# Autodesk Inventor assembly: YAxisMotorRight
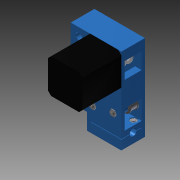
[picture p0: Inventor's stored thumbnail of the model, 180x180]
Saved by Autodesk Inventor 2015 SP1 (Build 190203100, 203)
## iProperties
Created: 2014-08-15
Part Number: YAxisMotorRight
Document SubType Name: Assembly
Designer: Jack
Mass: 240.117 g
Surface Area: 676.48 cm^2
Volume: 180.958 cm^3
Density: 1.32692 g/cm^3
Author: Jack
Title: Y Motor Right
## Documents named in this file (16)
- C:\Users\Jack\ownCloud\Projects\CrossBot\InventorModel\YAxis\YAxisMotorRight.iam
- C:\Users\Jack\ownCloud\Projects\CrossBot\InventorModel\YAxis\YAxisMotor\YMotorBlockRight.ipt
- C:\Users\Jack\ownCloud\Projects\CrossBot\InventorModel\YAxis\YAxisMotor\YMotorCapRight.ipt
- C:\Users\Jack\ownCloud\Projects\CrossBot\InventorModel\Hardware\Bolts\SHCS\SHCS4\SHCS4x30.ipt
- C:\Users\Jack\ownCloud\Projects\CrossBot\InventorModel\Hardware\Bolts\SHCS\SHCS3\SHCS3x8.ipt
- C:\Users\Jack\ownCloud\Projects\CrossBot\InventorModel\Hardware\Bearing\BearingRadialBall\BearingRadialBallF624zz.ipt
- C:\Users\Jack\ownCloud\Projects\CrossBot\InventorModel\Hardware\Wahsers\M4Washer.ipt
- C:\Users\Jack\ownCloud\Projects\CrossBot\InventorModel\Hardware\Nuts\Nut4.ipt
- C:\Users\Jack\ownCloud\Projects\CrossBot\InventorModel\Hardware\Bolts\SHCS\SHCS4\SHCS4x15.ipt
- C:\Users\Jack\ownCloud\Projects\CrossBot\InventorModel\YAxis\YAxisBearingSpacer.ipt
- C:\Users\Jack\ownCloud\Projects\CrossBot\InventorModel\Electronics\Motors\StepperMotorNema17x48mm.ipt
- C:\Users\Jack\ownCloud\Projects\CrossBot\InventorModel\Hardware\Belt\PulleyGT2x36x5Bore.ipt
- C:\Users\Jack\ownCloud\Projects\CrossBot\InventorModel\Hardware\Belt\GT2Idler.iam
- C:\Users\Jack\ownCloud\Projects\CrossBot\InventorModel\YAxis\YAxisBeltIdlerSpacer.ipt
- C:\Users\Jack\ownCloud\Projects\CrossBot\InventorModel\Hardware\Bolts\FHS\FHS4\FHS4x8.ipt
- C:\Users\Jack\ownCloud\Projects\CrossBot\InventorModel\Hardware\Bolts\SHCS\SHCS4\SHCS4x8.ipt
## Components (40 placed, 15 different names)
1. YMotorBlockRight:1 — Mate:5, Flush:3, Mate:4, Mate:1, Mate:10, Mate:7, Mate:9, Mate:8, Mate:18, Mate:12, Mate:16, Mate:13, Mate:17, Mate:14, Mate:15, Mate:11, Mate:48, Angle:1, Mate:50, Mate:52, Angle:3, Angle:2, Slider:2, Mate:74, Mate:76, Mate:80, Mate:84, Mate:94, Mate:95, Mate:96, Flush:3, Mate:101, Mate:109, Mate:110, Flush:4, Mate:111, Mate:112, Mate:113, Mate:114, Mate:115, Flush:5
2. YMotorCapRight:1 — Mate:1, Mate:86, Mate:87, Mate:88, Mate:89, Mate:90, Mate:91, Mate:92, Mate:93
3. YAxisBearingSpacer:2 — Mate:83, Mate:84
4. YAxisBearingSpacer:3 — Mate:79, Mate:80
5. SHCS4x15:1 — Mate:86, Mate:91
6. SHCS4x15:2 — Mate:88, Mate:92
7. SHCS4x15:3 — Mate:89, Mate:93
8. SHCS4x15:4 — Mate:87, Mate:90, Mate:106
9. StepperMotorNema17x48mm:1 — Mate:94, Mate:95, Mate:96, Mate:100
10. PulleyGT2x36x5Bore:1 — Mate:100, Flush:3
11. GT2Idler:1 [sub-assembly] — Mate:102, Mate:103, Mate:104
12. YAxisBeltIdlerSpacer:1 — Mate:107, Mate:108, Mate:109
13. FHS4x8:1 — Mate:110, Flush:4
14. SHCS4x8:1 — Mate:111, Mate:112
15. SHCS4x8:2 — Mate:113, Mate:114
16. FHS4x8:2 — Mate:115, Flush:5
17. BearingRadialBallF624zz:1 — Mate:24, Mate:23, Mate:26, Mate:25
18. BearingRadialBallF624zz:2 — Mate:24, Mate:23, Mate:28, Mate:27
19. BearingRadialBallF624zz:5 — Mate:40, Mate:39, Mate:42, Mate:41
20. BearingRadialBallF624zz:6 — Mate:40, Mate:39, Mate:44, Mate:43
21. M4Washer:3 — Mate:37, Mate:101, Mate:103
22. M4Washer:5 — Mate:45, Mate:42, Mate:41, Mate:76
23. Nut4:3 — Mate:52, Angle:3, Mate:51
24. Nut4:2 — Mate:50, Mate:49, Angle:2
25. Nut4:1 — Mate:48, Angle:1, Mate:47
26. M4Washer:6 — Mate:44, Mate:43
27. M4Washer:4 — Mate:104, Mate:105
28. M4Washer:2 — Mate:29, Mate:28, Mate:27
29. M4Washer:1 — Mate:26, Mate:25, Mate:74
30. SHCS4x30:2 — Mate:9, Mate:8, Mate:29, Mate:47, Mate:79
31. SHCS4x30:1 — Mate:10, Mate:7, Mate:37, Mate:49, Mate:102, Mate:105, Mate:107, Mate:108
32. SHCS4x30:3 — Mate:45, Mate:51, Slider:2, Mate:83
33. SHCS3x8:1 — Mate:18, Mate:12
34. SHCS3x8:4 — Mate:15, Mate:11
35. SHCS3x8:3 — Mate:17, Mate:14
36. SHCS3x8:2 — Mate:16, Mate:13
37. Nut4:4
38. Nut4:5
39. Nut4:7
40. Nut4:6 — Mate:106
## Relationships (77: Mate 70, Angle 3, Flush 3, TranslationJoint 1)
- Mate:5: YMotorBlockRight:1
- Flush:3 [Mate]: YMotorBlockRight:1
- Mate:4: YMotorBlockRight:1
- Mate:1: YMotorBlockRight:1 ↔ YMotorCapRight:1
- Mate:10: YMotorBlockRight:1 ↔ SHCS4x30:1
- Mate:7: YMotorBlockRight:1 ↔ SHCS4x30:1
- Mate:9: YMotorBlockRight:1 ↔ SHCS4x30:2
- Mate:8: YMotorBlockRight:1 ↔ SHCS4x30:2
- Mate:18: YMotorBlockRight:1 ↔ SHCS3x8:1
- Mate:12: YMotorBlockRight:1 ↔ SHCS3x8:1
- Mate:16: YMotorBlockRight:1 ↔ SHCS3x8:2
- Mate:13: YMotorBlockRight:1 ↔ SHCS3x8:2
- Mate:17: YMotorBlockRight:1 ↔ SHCS3x8:3
- Mate:14: YMotorBlockRight:1 ↔ SHCS3x8:3
- Mate:15: YMotorBlockRight:1 ↔ SHCS3x8:4
- Mate:11: YMotorBlockRight:1 ↔ SHCS3x8:4
- Mate:24: BearingRadialBallF624zz:1 ↔ BearingRadialBallF624zz:2
- Mate:23: BearingRadialBallF624zz:1 ↔ BearingRadialBallF624zz:2
- Mate:26: BearingRadialBallF624zz:1 ↔ M4Washer:1
- Mate:25: BearingRadialBallF624zz:1 ↔ M4Washer:1
- Mate:29: M4Washer:2 ↔ SHCS4x30:2
- Mate:28: BearingRadialBallF624zz:2 ↔ M4Washer:2
- Mate:27: BearingRadialBallF624zz:2 ↔ M4Washer:2
- Mate:37: M4Washer:3 ↔ SHCS4x30:1
- Mate:40: BearingRadialBallF624zz:5 ↔ BearingRadialBallF624zz:6
- Mate:39: BearingRadialBallF624zz:5 ↔ BearingRadialBallF624zz:6
- Mate:45: M4Washer:5 ↔ SHCS4x30:3
- Mate:42: BearingRadialBallF624zz:5 ↔ M4Washer:5
- Mate:41: BearingRadialBallF624zz:5 ↔ M4Washer:5
- Mate:44: BearingRadialBallF624zz:6 ↔ M4Washer:6
- Mate:43: BearingRadialBallF624zz:6 ↔ M4Washer:6
- Mate:48: YMotorBlockRight:1 ↔ Nut4:1
- Angle:1 (0 deg): YMotorBlockRight:1 ↔ Nut4:1
- Mate:47: Nut4:1 ↔ SHCS4x30:2
- Mate:50: YMotorBlockRight:1 ↔ Nut4:2
- Mate:49: Nut4:2 ↔ SHCS4x30:1
- Mate:52: YMotorBlockRight:1 ↔ Nut4:3
- Angle:3 (0 deg): YMotorBlockRight:1 ↔ Nut4:3
- Mate:51: Nut4:3 ↔ SHCS4x30:3
- Angle:2 (0 deg): YMotorBlockRight:1 ↔ Nut4:2
- Slider:2 [TranslationJoint]: YMotorBlockRight:1 ↔ SHCS4x30:3
- Mate:74: YMotorBlockRight:1 ↔ M4Washer:1
- Mate:76: YMotorBlockRight:1 ↔ M4Washer:5
- Mate:79: YAxisBearingSpacer:3 ↔ SHCS4x30:2
- Mate:80: YMotorBlockRight:1 ↔ YAxisBearingSpacer:3
- Mate:83: YAxisBearingSpacer:2 ↔ SHCS4x30:3
- Mate:84: YMotorBlockRight:1 ↔ YAxisBearingSpacer:2
- Mate:86: YMotorCapRight:1 ↔ SHCS4x15:1
- Mate:87: YMotorCapRight:1 ↔ SHCS4x15:4
- Mate:88: YMotorCapRight:1 ↔ SHCS4x15:2
- Mate:89: YMotorCapRight:1 ↔ SHCS4x15:3
- Mate:90: YMotorCapRight:1 ↔ SHCS4x15:4
- Mate:91: YMotorCapRight:1 ↔ SHCS4x15:1
- Mate:92: YMotorCapRight:1 ↔ SHCS4x15:2
- Mate:93: YMotorCapRight:1 ↔ SHCS4x15:3
- Mate:94: YMotorBlockRight:1 ↔ StepperMotorNema17x48mm:1
- Mate:95: YMotorBlockRight:1 ↔ StepperMotorNema17x48mm:1
- Mate:96: YMotorBlockRight:1 ↔ StepperMotorNema17x48mm:1
- Mate:100: StepperMotorNema17x48mm:1 ↔ PulleyGT2x36x5Bore:1
- Flush:3 (-11.95 mm): YMotorBlockRight:1 ↔ PulleyGT2x36x5Bore:1
- Mate:101: YMotorBlockRight:1 ↔ M4Washer:3
- Mate:102: GT2Idler:1 ↔ SHCS4x30:1
- Mate:103: GT2Idler:1 ↔ M4Washer:3
- Mate:104: GT2Idler:1 ↔ M4Washer:4
- Mate:105: M4Washer:4 ↔ SHCS4x30:1
- Mate:106: SHCS4x15:4 ↔ Nut4:6
- Mate:107: YAxisBeltIdlerSpacer:1 ↔ SHCS4x30:1
- Mate:108: YAxisBeltIdlerSpacer:1 ↔ SHCS4x30:1
- Mate:109: YMotorBlockRight:1 ↔ YAxisBeltIdlerSpacer:1
- Mate:110: YMotorBlockRight:1 ↔ FHS4x8:1
- Flush:4: YMotorBlockRight:1 ↔ FHS4x8:1
- Mate:111: YMotorBlockRight:1 ↔ SHCS4x8:1
- Mate:112: YMotorBlockRight:1 ↔ SHCS4x8:1
- Mate:113: YMotorBlockRight:1 ↔ SHCS4x8:2
- Mate:114: YMotorBlockRight:1 ↔ SHCS4x8:2
- Mate:115: YMotorBlockRight:1 ↔ FHS4x8:2
- Flush:5: YMotorBlockRight:1 ↔ FHS4x8:2
